# Autodesk Inventor assembly: Cadena 428
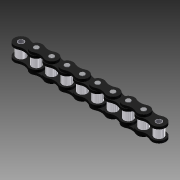
[picture p0: Inventor's stored thumbnail of the model, 180x180]
Saved by Autodesk Inventor 2012 (Build 160160000, 160)
## iProperties
Created: 2011-08-31
Part Number: Cadena 428
Document SubType Name: Assembly
Designer: Luis
Author: Luis
## Documents named in this file (4)
- H:\Cadena 428\Cadena 428.iam
- H:\Cadena 428\Eslabon interno.iam
- H:\Cadena 428\Gancho.iam
- H:\Cadena 428\Concha1.ipt
## Components (13 placed, 3 different names)
1. Gancho:1 [sub-assembly] — Insert:1, Insert:2
2. Gancho:2 [sub-assembly] — Insert:3, Insert:4
3. Gancho:3 [sub-assembly] — Insert:5, Insert:6
4. Gancho:4 [sub-assembly] — Insert:7, Insert:8
5. Eslabon interno:1 [sub-assembly] — Insert:2, Insert:3, Insert:10
6. Eslabon interno:2 [sub-assembly] — Insert:4, Insert:5, Insert:11
7. Eslabon interno:3 [sub-assembly] — Insert:6, Insert:7, Insert:12
8. Eslabon interno:4 [sub-assembly] — Insert:1, Insert:9
9. Eslabon interno:5 [sub-assembly] — Insert:8
10. Concha1:1 — Insert:9
11. Concha1:2 — Insert:10
12. Concha1:3 — Insert:11
13. Concha1:4 — Insert:12
## Relationships (12: Insert 12)
- Insert:1: Gancho:1 ↔ Eslabon interno:4
- Insert:2: Gancho:1 ↔ Eslabon interno:1
- Insert:3: Gancho:2 ↔ Eslabon interno:1
- Insert:4: Gancho:2 ↔ Eslabon interno:2
- Insert:5: Gancho:3 ↔ Eslabon interno:2
- Insert:6: Gancho:3 ↔ Eslabon interno:3
- Insert:7: Gancho:4 ↔ Eslabon interno:3
- Insert:8: Gancho:4 ↔ Eslabon interno:5
- Insert:9: Eslabon interno:4 ↔ Concha1:1
- Insert:10: Eslabon interno:1 ↔ Concha1:2
- Insert:11: Eslabon interno:2 ↔ Concha1:3
- Insert:12: Eslabon interno:3 ↔ Concha1:4
